# Autodesk Inventor assembly: cap
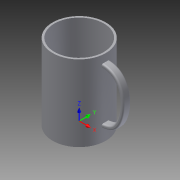
[picture p0: Inventor's stored thumbnail of the model, 180x180]
Saved by Autodesk Inventor 2014 (Build 180170000, 170)
## iProperties
Created: 2014-07-25
Part Number: cap
Document SubType Name: Assembly
Designer: hatakeyama
Author: hatakeyama
## Documents named in this file (2)
- C:\Users\hatakeyama\Desktop\workspace\cap.iam
- C:\Users\hatakeyama\Desktop\homeroom\インポートされたコンポーネント\cap\cap.ipt
## Components (1 placed, 1 different names)
1. cap:1 — メイト:1, メイト:2
## Relationships (2: Mate 2)
- メイト:1 [Mate]: cap:1
- メイト:2 [Mate]: cap:1
